# Autodesk Inventor assembly: Top Cover Assembly
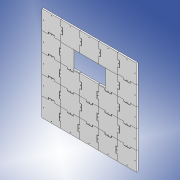
[picture p0: Inventor's stored thumbnail of the model, 180x180]
Saved by Autodesk Inventor 2017 SP1 (Build 210196100, 196)
## iProperties
Created: 2017-08-15
Part Number: Top Cover Assembly
Document SubType Name: Assembly
Designer: Zach
Author: Zach
## Documents named in this file (9)
- C:\Users\Zach\Documents\GitHub\cr-laundry-robot\src\Base\Top Cover Assembly\Top Cover Assembly.iam
- C:\Users\Zach\Documents\GitHub\cr-laundry-robot\src\Base\Top Cover Assembly\TC001.ipt
- C:\Users\Zach\Documents\GitHub\cr-laundry-robot\src\Base\Top Cover Assembly\TA002.ipt
- C:\Users\Zach\Documents\GitHub\cr-laundry-robot\src\Base\Top Cover Assembly\TC003.ipt
- C:\Users\Zach\Documents\GitHub\cr-laundry-robot\src\Base\Top Cover Assembly\TC004.ipt
- C:\Users\Zach\Documents\GitHub\cr-laundry-robot\src\Base\Top Cover Assembly\TC005.ipt
- C:\Users\Zach\Documents\GitHub\cr-laundry-robot\src\Base\Top Cover Assembly\TC006.ipt
- C:\Users\Zach\Documents\GitHub\cr-laundry-robot\src\Base\Top Cover Assembly\TC007.ipt
- C:\Users\Zach\Documents\GitHub\cr-laundry-robot\src\Base\Top Cover Assembly\TC008.ipt
## Components (24 placed, 8 different names)
1. TC001:1 — Mate:1, Mate:2, Mate:15, Mate:16
2. TA002:1 — Mate:1, Mate:2, Mate:3, Mate:5, Mate:54
3. TA002:2 — Mate:3, Mate:4, Mate:5, Mate:6, Mate:62
4. TA002:3 — Mate:4, Mate:6, Mate:7, Mate:8, Mate:61
5. TC001:2 — Mate:7, Mate:8, Mate:36, Mate:37
6. TC001:3 — Mate:41, Mate:45
7. TA002:4 — Mate:50, Flush:7
8. TA002:5 — Mate:57, Flush:5
9. TA002:6 — Mate:15, Mate:16, Mate:55, Flush:6
10. TC001:4 — Mate:34, Mate:35, Mate:38, Mate:46
11. TA002:13 — Flush:1, Mate:36, Mate:37, Mate:60, Flush:4
12. TA002:14 — Flush:1, Flush:2, Mate:52, Flush:3
13. TA002:15 — Flush:2, Mate:34, Mate:35, Mate:42
14. TC003:1 — Mate:38, Mate:40, Mate:44, Mate:46, Mate:47, Flush:8
15. TC003:2 — Mate:40, Mate:43, Mate:44, Mate:47, Mate:48
16. TC003:3 — Mate:41, Mate:43, Mate:45, Mate:48
17. TC004:1 — Mate:42, Mate:53, Flush:8
18. TC005:1 — Mate:50, Mate:58, Flush:7
19. TC006:1 — Mate:52, Mate:53, Mate:59, Flush:3
20. TC006:2 — Mate:56, Mate:57, Mate:58, Flush:5, Mate:65
21. TC006:3 — Mate:59, Mate:60, Mate:61, Flush:4, Mate:63
22. TC006:4 — Mate:54, Mate:55, Mate:56, Flush:6, Flush:9
23. TC007:1 — Mate:62, Mate:63, Flush:9, Mate:64, Flush:10
24. TC008:1 — Mate:64, Flush:10, Mate:65
## Relationships (59: Mate 49, Flush 10)
- Mate:1: TC001:1 ↔ TA002:1
- Mate:2: TC001:1 ↔ TA002:1
- Mate:3: TA002:1 ↔ TA002:2
- Mate:4: TA002:2 ↔ TA002:3
- Mate:5: TA002:1 ↔ TA002:2
- Mate:6: TA002:2 ↔ TA002:3
- Mate:7: TA002:3 ↔ TC001:2
- Mate:8: TA002:3 ↔ TC001:2
- [Mate]: TC001:3 ↔ TA002:4
- [Mate]: TC001:3 ↔ TA002:4
- [Mate]: TA002:4 ↔ TA002:5
- [Mate]: TA002:5 ↔ TA002:6
- [Mate]: TA002:4 ↔ TA002:5
- [Mate]: TA002:5 ↔ TA002:6
- Mate:15: TC001:1 ↔ TA002:6
- Mate:16: TC001:1 ↔ TA002:6
- [Mate]: TA002:13 ↔ TA002:14
- [Mate]: TA002:14 ↔ TA002:15
- [Mate]: TA002:13 ↔ TA002:14
- [Mate]: TA002:14 ↔ TA002:15
- Flush:1: TA002:13 ↔ TA002:14
- Flush:2: TA002:14 ↔ TA002:15
- Mate:34: TC001:4 ↔ TA002:15
- Mate:35: TC001:4 ↔ TA002:15
- Mate:36: TC001:2 ↔ TA002:13
- Mate:37: TC001:2 ↔ TA002:13
- Mate:38: TC001:4 ↔ TC003:1
- Mate:40: TC003:1 ↔ TC003:2
- Mate:41: TC001:3 ↔ TC003:3
- Mate:42: TA002:15 ↔ TC004:1
- Mate:43: TC003:2 ↔ TC003:3
- Mate:44: TC003:1 ↔ TC003:2
- Mate:45: TC001:3 ↔ TC003:3
- Mate:46: TC001:4 ↔ TC003:1
- Mate:47: TC003:1 ↔ TC003:2
- Mate:48: TC003:2 ↔ TC003:3
- Mate:50: TA002:4 ↔ TC005:1
- Mate:52: TA002:14 ↔ TC006:1
- Mate:53: TC004:1 ↔ TC006:1
- Mate:54: TA002:1 ↔ TC006:4
- Mate:55: TA002:6 ↔ TC006:4
- Mate:56: TC006:2 ↔ TC006:4
- Mate:57: TA002:5 ↔ TC006:2
- Mate:58: TC005:1 ↔ TC006:2
- Mate:59: TC006:1 ↔ TC006:3
- Mate:60: TA002:13 ↔ TC006:3
- Mate:61: TA002:3 ↔ TC006:3
- Flush:3: TA002:14 ↔ TC006:1
- Flush:4: TA002:13 ↔ TC006:3
- Flush:5: TA002:5 ↔ TC006:2
- Flush:6: TA002:6 ↔ TC006:4
- Flush:7: TA002:4 ↔ TC005:1
- Flush:8: TC003:1 ↔ TC004:1
- Mate:62: TA002:2 ↔ TC007:1
- Mate:63: TC006:3 ↔ TC007:1
- Flush:9: TC006:4 ↔ TC007:1
- Mate:64: TC007:1 ↔ TC008:1
- Flush:10: TC007:1 ↔ TC008:1
- Mate:65: TC006:2 ↔ TC008:1
## Named parameters: d8_d0 = 0 mm, d9_d1 = 0 mm, d10_d2 = 0 mm, d11_d3 = 0 mm, d12_d4 = 0 mm, d13_d5 = 0 mm, d29_d10_d2 = 0 mm, d30_d11_d3 = 0 mm, d31_d12_d4 = 0 mm, d32_d13_d5 = 0 mm
